# Autodesk Inventor assembly: Alpha Motor Assembly
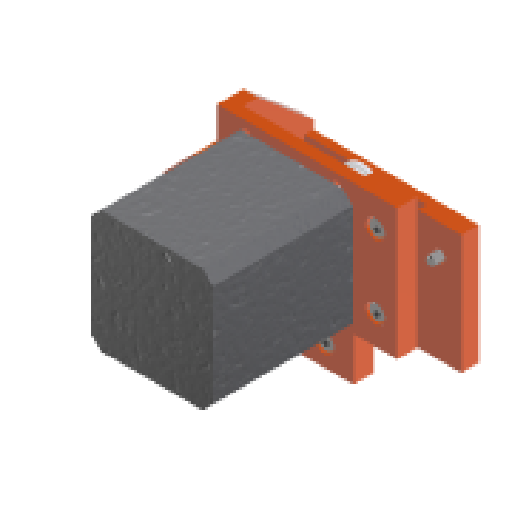
[picture p0: Inventor's stored thumbnail of the model, 512x512]
Saved by Autodesk Inventor 2023.2 (Build 272271000, 271)
## iProperties
Created: 2023-02-03
Part Number: Alpha Motor Assembly
Document SubType Name: Assembly
Designer: remop
Author: remop
## Documents named in this file (8)
- C:\Users\remop\OneDrive\Documents\Inventor\3D Printers\LuEVO\Mk5_FullKinematic\Alpha Motor Assembly.iam
- C:\Users\remop\OneDrive\Documents\Inventor\3D Printers\LuEVO\Mk5_FullKinematic\Alpha Motor Mount.ipt
- C:\Users\remop\OneDrive\Documents\Inventor\3D Printers\LuEVO\Mk5_FullKinematic\XY Axis Motor (Stepper).ipt
- C:\Users\remop\OneDrive\Documents\Inventor\3D Printers\LuEVO\Mk1\Belt_Pulley_20T.ipt
- C:\Users\remop\OneDrive\Documents\Inventor\3D Printers\LuEVO\Mk5_FullKinematic\Beta Idler Top.ipt
- C:\Users\remop\OneDrive\Documents\Inventor\Content Center Files\R2023\en-US\AS 1420\AS 1420 - 1973 - M3 x 6.ipt
- C:\Users\remop\OneDrive\Documents\Inventor\Content Center Files\R2023\en-US\AS 1420\AS 1420 - 1973 - M3 x 12.ipt
- C:\Users\remop\OneDrive\Documents\Inventor\Content Center Files\R2023\en-US\BS 4168(6)\BS 4168 - M4 x 8(6).ipt
## Components (18 placed, 7 different names)
1. Alpha Motor Mount:1 — Flush:1, Flush:2, Mate:1, Rigid:1, Insert:5, Insert:7, Insert:9, Insert:11, Insert:12, Insert:13, Insert:14, Insert:15
2. XY Axis Motor (Stepper):1 — Rigid:1, Rigid:2
3. Belt_Pulley_20T:1 — Rigid:2
4. Beta Idler Top:1 — Flush:1, Flush:2, Mate:1, Insert:1, Insert:2, Insert:3, Insert:4, Insert:16, Insert:17
5. AS 1420 - Metric M3 x 6:1 — Insert:1
6. AS 1420 - Metric M3 x 6:2 — Insert:2
7. AS 1420 - Metric M3 x 6:3 — Insert:3
8. AS 1420 - Metric M3 x 12:1 — Insert:4
9. AS 1420 - Metric M3 x 6:4 — Insert:5
10. AS 1420 - Metric M3 x 6:6 — Insert:7
11. AS 1420 - Metric M3 x 6:8 — Insert:9
12. AS 1420 - Metric M3 x 6:10 — Insert:11
13. AS 1420 - Metric M3 x 6:11 — Insert:12
14. AS 1420 - Metric M3 x 6:12 — Insert:13
15. AS 1420 - Metric M3 x 6:13 — Insert:14
16. AS 1420 - Metric M3 x 6:14 — Insert:15
17. BS 4168 : Part 6 Hexagon socket countersunk and button head screws - Metric series - Metric M4 x 8:1 — Insert:16
18. BS 4168 : Part 6 Hexagon socket countersunk and button head screws - Metric series - Metric M4 x 8:2 — Insert:17
## Relationships (19: Insert 14, Flush 2, WeldJoint 2, Mate 1)
- Flush:1: Alpha Motor Mount:1 ↔ Beta Idler Top:1
- Flush:2: Alpha Motor Mount:1 ↔ Beta Idler Top:1
- Mate:1 (15 mm): Alpha Motor Mount:1 ↔ Beta Idler Top:1
- Rigid:1 [WeldJoint]: Alpha Motor Mount:1 ↔ XY Axis Motor (Stepper):1
- Rigid:2 [WeldJoint] (-0.5 mm): XY Axis Motor (Stepper):1 ↔ Belt_Pulley_20T:1
- Insert:1: Beta Idler Top:1 ↔ AS 1420 - Metric M3 x 6:1
- Insert:2: Beta Idler Top:1 ↔ AS 1420 - Metric M3 x 6:2
- Insert:3: Beta Idler Top:1 ↔ AS 1420 - Metric M3 x 6:3
- Insert:4: Beta Idler Top:1 ↔ AS 1420 - Metric M3 x 12:1
- Insert:5: Alpha Motor Mount:1 ↔ AS 1420 - Metric M3 x 6:4
- Insert:7: Alpha Motor Mount:1 ↔ AS 1420 - Metric M3 x 6:6
- Insert:9: Alpha Motor Mount:1 ↔ AS 1420 - Metric M3 x 6:8
- Insert:11: Alpha Motor Mount:1 ↔ AS 1420 - Metric M3 x 6:10
- Insert:12: Alpha Motor Mount:1 ↔ AS 1420 - Metric M3 x 6:11
- Insert:13: Alpha Motor Mount:1 ↔ AS 1420 - Metric M3 x 6:12
- Insert:14: Alpha Motor Mount:1 ↔ AS 1420 - Metric M3 x 6:13
- Insert:15: Alpha Motor Mount:1 ↔ AS 1420 - Metric M3 x 6:14
- Insert:16: Beta Idler Top:1 ↔ BS 4168 : Part 6 Hexagon socket countersunk and button head screws - Metric series - Metric M4 x 8:1
- Insert:17: Beta Idler Top:1 ↔ BS 4168 : Part 6 Hexagon socket countersunk and button head screws - Metric series - Metric M4 x 8:2
